# Autodesk Inventor assembly: Rear-Bed-Holder
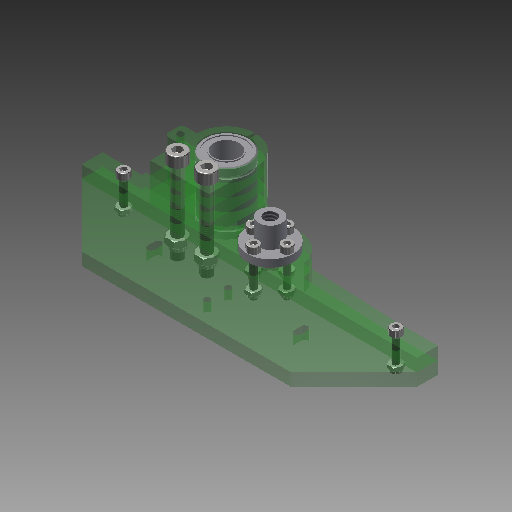
[picture p0: Inventor's stored thumbnail of the model, 512x512]
Saved by Autodesk Inventor 2017 (Build 210142000, 142)
## iProperties
Created: 2016-07-12
Part Number: Rear-Bed-Holder
Document SubType Name: Assembly
Designer: joshmamo
Author: joshmamo
## Documents named in this file (11)
- C:\All INVENTOR\SL-Inventor\SL-Beast 3D Printer\Rear-Bed-Holder.iam
- C:\All INVENTOR\SL-Inventor\SL-Beast 3D Printer\en-US\ANSI B18.3.1M(6)\ANSI B18.3.1M - M5x0.8 x 40(1).ipt
- C:\All INVENTOR\SL-Inventor\SL-Beast 3D Printer\en-US\ANSI B18.3.1M(6)\ANSI B18.3.1M - M3x0.5 x 16(1).ipt
- C:\All INVENTOR\SL-Inventor\SL-Beast 3D Printer\en-US\ANSI B18.16.3M(2)\ANSI B18.16.3M - Property Class 5 and 10 - Metric M3 x 0.5 Metal Type.ipt
- C:\All INVENTOR\SL-Inventor\SL-Beast 3D Printer\en-US\ANSI B18.16.3M(2)\ANSI B18.16.3M - Property Class 9 - Metric M5 x 0.8 Metal Type.ipt
- C:\All INVENTOR\SL-Inventor\SL-Beast 3D Printer\en-US\ANSI B18.3.1M(6)\ANSI B18.3.1M - M3x0.5 x 20(1).ipt
- C:\All INVENTOR\SL-Inventor\SL-Beast 3D Printer\Rear-Bed-Holder-Lower_MIR.ipt
- C:\All INVENTOR\SL-Inventor\SL-Beast 3D Printer\Rear-Bed-Holder-mid_MIR.ipt
- C:\All INVENTOR\SL-Inventor\SL-Beast 3D Printer\Left Bed Holder Upper_MIR1.ipt
- C:\All INVENTOR\SL-Inventor\SL-Beast 3D Printer\Brass-Nut_MIR1.ipt
- C:\All INVENTOR\SL-Inventor\SL-Beast 3D Printer\LM12UU_MIR1.ipt
## Components (25 placed, 10 different names)
1. Rear-Bed-Holder-Lower_MIR:1 — Flush:11, Flush:12, Mate:44, Mate:45, Mate:57, Mate:59, Mate:61, Mate:63, Mate:67, Mate:69, Mate:71, Mate:73, Flush:19
2. Rear-Bed-Holder-mid_MIR:1 — Flush:11, Flush:12, Mate:44, Mate:45, Flush:13, Flush:14, Mate:46, Mate:49, Mate:50, Mate:51, Mate:52, Mate:53, Mate:54, Mate:55, Mate:56, Mate:65, Mate:66
3. Left Bed Holder Upper_MIR1:1 — Flush:13, Flush:14, Mate:46, Flush:15, Flush:16, Mate:47
4. Left Bed Holder Upper_MIR1:2 — Flush:15, Flush:16, Mate:47, Mate:48, Flush:17, Flush:18
5. Left Bed Holder Upper_MIR1:3 — Mate:48, Flush:17, Flush:18, Insert:7, Insert:8, Mate:75
6. Forged Socket Head Cap Screw - Metric M5x0.8 x 40:3 — Insert:7, Mate:64
7. Forged Socket Head Cap Screw - Metric M5x0.8 x 40:4 — Insert:8, Mate:62
8. Forged Socket Head Cap Screw - Metric M3x0.5 x 16:8 — Mate:49, Mate:50
9. Forged Socket Head Cap Screw - Metric M3x0.5 x 16:9 — Mate:51, Mate:52, Mate:58
10. Forged Socket Head Cap Screw - Metric M3x0.5 x 16:10 — Mate:53, Mate:54
11. Forged Socket Head Cap Screw - Metric M3x0.5 x 16:11 — Mate:55, Mate:56, Mate:60
12. Prevailing Torque Type Hex Nut - Steel Metric Property Class 5 and 10 - Metric M3 x 0.5 Metal Type:10 — Mate:57, Mate:58
13. Prevailing Torque Type Hex Nut - Steel Metric Property Class 5 and 10 - Metric M3 x 0.5 Metal Type:11 — Mate:59, Mate:60
14. Prevailing Torque Type Hex Nut - Steel Metric Property Class 9 - Metric M5 x 0.8 Metal Type:3 — Mate:61, Mate:62
15. Prevailing Torque Type Hex Nut - Steel Metric Property Class 9 - Metric M5 x 0.8 Metal Type:4 — Mate:63, Mate:64
16. Brass-Nut_MIR1:1 — Mate:65, Mate:66, Insert:9, Insert:10, Insert:11, Insert:12
17. Forged Socket Head Cap Screw - Metric M3x0.5 x 20:5 — Insert:9, Mate:68
18. Forged Socket Head Cap Screw - Metric M3x0.5 x 20:6 — Insert:10, Mate:74
19. Forged Socket Head Cap Screw - Metric M3x0.5 x 20:7 — Insert:11, Mate:70
20. Forged Socket Head Cap Screw - Metric M3x0.5 x 20:8 — Insert:12, Mate:72
21. Prevailing Torque Type Hex Nut - Steel Metric Property Class 5 and 10 - Metric M3 x 0.5 Metal Type:12 — Mate:67, Mate:68
22. Prevailing Torque Type Hex Nut - Steel Metric Property Class 5 and 10 - Metric M3 x 0.5 Metal Type:13 — Mate:69, Mate:70
23. Prevailing Torque Type Hex Nut - Steel Metric Property Class 5 and 10 - Metric M3 x 0.5 Metal Type:14 — Mate:71, Mate:72
24. Prevailing Torque Type Hex Nut - Steel Metric Property Class 5 and 10 - Metric M3 x 0.5 Metal Type:15 — Mate:73, Mate:74
25. LM12UU_MIR1:1 — Flush:19, Mate:75
## Relationships (47: Mate 32, Flush 9, Insert 6)
- Flush:11: Rear-Bed-Holder-Lower_MIR:1 ↔ Rear-Bed-Holder-mid_MIR:1
- Flush:12: Rear-Bed-Holder-Lower_MIR:1 ↔ Rear-Bed-Holder-mid_MIR:1
- Mate:44: Rear-Bed-Holder-Lower_MIR:1 ↔ Rear-Bed-Holder-mid_MIR:1
- Mate:45: Rear-Bed-Holder-Lower_MIR:1 ↔ Rear-Bed-Holder-mid_MIR:1
- Flush:13: Rear-Bed-Holder-mid_MIR:1 ↔ Left Bed Holder Upper_MIR1:1
- Flush:14: Rear-Bed-Holder-mid_MIR:1 ↔ Left Bed Holder Upper_MIR1:1
- Mate:46: Rear-Bed-Holder-mid_MIR:1 ↔ Left Bed Holder Upper_MIR1:1
- Flush:15: Left Bed Holder Upper_MIR1:1 ↔ Left Bed Holder Upper_MIR1:2
- Flush:16: Left Bed Holder Upper_MIR1:1 ↔ Left Bed Holder Upper_MIR1:2
- Mate:47: Left Bed Holder Upper_MIR1:1 ↔ Left Bed Holder Upper_MIR1:2
- Mate:48: Left Bed Holder Upper_MIR1:2 ↔ Left Bed Holder Upper_MIR1:3
- Flush:17: Left Bed Holder Upper_MIR1:2 ↔ Left Bed Holder Upper_MIR1:3
- Flush:18: Left Bed Holder Upper_MIR1:2 ↔ Left Bed Holder Upper_MIR1:3
- Insert:7: Left Bed Holder Upper_MIR1:3 ↔ Forged Socket Head Cap Screw - Metric M5x0.8 x 40:3
- Insert:8: Left Bed Holder Upper_MIR1:3 ↔ Forged Socket Head Cap Screw - Metric M5x0.8 x 40:4
- Mate:49: Rear-Bed-Holder-mid_MIR:1 ↔ Forged Socket Head Cap Screw - Metric M3x0.5 x 16:8
- Mate:50: Rear-Bed-Holder-mid_MIR:1 ↔ Forged Socket Head Cap Screw - Metric M3x0.5 x 16:8
- Mate:51: Rear-Bed-Holder-mid_MIR:1 ↔ Forged Socket Head Cap Screw - Metric M3x0.5 x 16:9
- Mate:52: Rear-Bed-Holder-mid_MIR:1 ↔ Forged Socket Head Cap Screw - Metric M3x0.5 x 16:9
- Mate:53: Rear-Bed-Holder-mid_MIR:1 ↔ Forged Socket Head Cap Screw - Metric M3x0.5 x 16:10
- Mate:54: Rear-Bed-Holder-mid_MIR:1 ↔ Forged Socket Head Cap Screw - Metric M3x0.5 x 16:10
- Mate:55: Rear-Bed-Holder-mid_MIR:1 ↔ Forged Socket Head Cap Screw - Metric M3x0.5 x 16:11
- Mate:56: Rear-Bed-Holder-mid_MIR:1 ↔ Forged Socket Head Cap Screw - Metric M3x0.5 x 16:11
- Mate:57: Rear-Bed-Holder-Lower_MIR:1 ↔ Prevailing Torque Type Hex Nut - Steel Metric Property Class 5 and 10 - Metric M3 x 0.5 Metal Type:10
- Mate:58: Forged Socket Head Cap Screw - Metric M3x0.5 x 16:9 ↔ Prevailing Torque Type Hex Nut - Steel Metric Property Class 5 and 10 - Metric M3 x 0.5 Metal Type:10
- Mate:59: Rear-Bed-Holder-Lower_MIR:1 ↔ Prevailing Torque Type Hex Nut - Steel Metric Property Class 5 and 10 - Metric M3 x 0.5 Metal Type:11
- Mate:60: Forged Socket Head Cap Screw - Metric M3x0.5 x 16:11 ↔ Prevailing Torque Type Hex Nut - Steel Metric Property Class 5 and 10 - Metric M3 x 0.5 Metal Type:11
- Mate:61: Rear-Bed-Holder-Lower_MIR:1 ↔ Prevailing Torque Type Hex Nut - Steel Metric Property Class 9 - Metric M5 x 0.8 Metal Type:3
- Mate:62: Forged Socket Head Cap Screw - Metric M5x0.8 x 40:4 ↔ Prevailing Torque Type Hex Nut - Steel Metric Property Class 9 - Metric M5 x 0.8 Metal Type:3
- Mate:63: Rear-Bed-Holder-Lower_MIR:1 ↔ Prevailing Torque Type Hex Nut - Steel Metric Property Class 9 - Metric M5 x 0.8 Metal Type:4
- Mate:64: Forged Socket Head Cap Screw - Metric M5x0.8 x 40:3 ↔ Prevailing Torque Type Hex Nut - Steel Metric Property Class 9 - Metric M5 x 0.8 Metal Type:4
- Mate:65: Rear-Bed-Holder-mid_MIR:1 ↔ Brass-Nut_MIR1:1
- Mate:66: Rear-Bed-Holder-mid_MIR:1 ↔ Brass-Nut_MIR1:1
- Insert:9: Brass-Nut_MIR1:1 ↔ Forged Socket Head Cap Screw - Metric M3x0.5 x 20:5
- Insert:10: Brass-Nut_MIR1:1 ↔ Forged Socket Head Cap Screw - Metric M3x0.5 x 20:6
- Insert:11: Brass-Nut_MIR1:1 ↔ Forged Socket Head Cap Screw - Metric M3x0.5 x 20:7
- Insert:12: Brass-Nut_MIR1:1 ↔ Forged Socket Head Cap Screw - Metric M3x0.5 x 20:8
- Mate:67: Rear-Bed-Holder-Lower_MIR:1 ↔ Prevailing Torque Type Hex Nut - Steel Metric Property Class 5 and 10 - Metric M3 x 0.5 Metal Type:12
- Mate:68: Forged Socket Head Cap Screw - Metric M3x0.5 x 20:5 ↔ Prevailing Torque Type Hex Nut - Steel Metric Property Class 5 and 10 - Metric M3 x 0.5 Metal Type:12
- Mate:69: Rear-Bed-Holder-Lower_MIR:1 ↔ Prevailing Torque Type Hex Nut - Steel Metric Property Class 5 and 10 - Metric M3 x 0.5 Metal Type:13
- Mate:70: Forged Socket Head Cap Screw - Metric M3x0.5 x 20:7 ↔ Prevailing Torque Type Hex Nut - Steel Metric Property Class 5 and 10 - Metric M3 x 0.5 Metal Type:13
- Mate:71: Rear-Bed-Holder-Lower_MIR:1 ↔ Prevailing Torque Type Hex Nut - Steel Metric Property Class 5 and 10 - Metric M3 x 0.5 Metal Type:14
- Mate:72: Forged Socket Head Cap Screw - Metric M3x0.5 x 20:8 ↔ Prevailing Torque Type Hex Nut - Steel Metric Property Class 5 and 10 - Metric M3 x 0.5 Metal Type:14
- Mate:73: Rear-Bed-Holder-Lower_MIR:1 ↔ Prevailing Torque Type Hex Nut - Steel Metric Property Class 5 and 10 - Metric M3 x 0.5 Metal Type:15
- Mate:74: Forged Socket Head Cap Screw - Metric M3x0.5 x 20:6 ↔ Prevailing Torque Type Hex Nut - Steel Metric Property Class 5 and 10 - Metric M3 x 0.5 Metal Type:15
- Flush:19: Rear-Bed-Holder-Lower_MIR:1 ↔ LM12UU_MIR1:1
- Mate:75: Left Bed Holder Upper_MIR1:3 ↔ LM12UU_MIR1:1
